# Autodesk Inventor assembly: Gripper
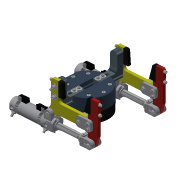
[picture p0: Inventor's stored thumbnail of the model, 180x180]
Saved by Autodesk Inventor 2020.1 (Build 241239000, 239)
## iProperties
Created: 2006-01-31
Part Number: Gripper
Document SubType Name: Assembly
Designer: Kevin
Manufacturer: Standard
Standards Organization: Custom
Weld Material: Default
Author: Kevin
Revision Number: -
## Documents named in this file (10)
- C:\Users\thomastremblay\Desktop\Inventor ACP Data\Gripper - References.iam
- C:\Users\thomastremblay\Desktop\Inventor ACP Data\Parts\210-100b.ipt
- C:\Users\thomastremblay\Desktop\Inventor ACP Data\Parts\210-101b.ipt
- C:\Users\thomastremblay\Desktop\Inventor ACP Data\Content Center\en-US\ISO 4762\M8-65.ipt
- C:\Users\thomastremblay\Desktop\Inventor ACP Data\Content Center\en-US\ISO 4762\M6-45.ipt
- C:\Users\thomastremblay\Desktop\Inventor ACP Data\Content Center\en-US\ISO 7089\10.ipt
- C:\Users\thomastremblay\Desktop\Inventor ACP Data\Content Center\en-US\ISO 4762\M8-30.ipt
- C:\Users\thomastremblay\Desktop\Inventor ACP Data\Parts\210-102 fb.ipt
- C:\Users\thomastremblay\Desktop\Inventor ACP Data\Assemblies\Clamp Assembly.iam
- C:\Users\thomastremblay\Desktop\Inventor ACP Data\Libraries\Simulation\Gripper_res_{3E676F27-C720-4572-8F7D-DA90B4A1A400}.fres
## Components (28 placed, 8 different names)
1. 210-100b:1 — Mate:1, Insert:1
2. 210-101b:1 — Mate:1, Insert:1, Mate:2, Mate:6, Mate:25, Mate:26, Mate:27, Mate:28, Mate:29, Insert:21, Mate:36, Mate:37, Mate:38, Mate:3
3. 210-102 fb:1 — Mate:2, Mate:3, Mate:42
4. 210-102 fb:2 — Mate:25, Mate:26, Mate:29, Mate:41, Rigid:1
5. Clamp Assembly:1 [sub-assembly]
6. Clamp Assembly:2 [sub-assembly] — Rigid:1
7. ISO 4762 M8 x 45:1 — Mate:6, Insert:22, Mate:42
8. ISO 7089 10 - 140 HV:1 — Insert:22
9. ISO 7089 10 - 140 HV:2 — Insert:23
10. ISO 4762 M8 x 45:2 — Insert:23, Mate:36
11. ISO 7089 10 - 140 HV:3 — Mate:28, Insert:25
12. ISO 4762 M8 x 45:3 — Insert:25, Mate:38
13. ISO 7089 10 - 140 HV:4 — Mate:27, Insert:24
14. ISO 4762 M8 x 45:4 — Mate:37, Insert:24
15. ISO 7089 10 - 140 HV:5 — Insert:33
16. ISO 7089 10 - 140 HV:6 — Insert:32
17. ISO 7089 10 - 140 HV:7 — Insert:28
18. ISO 7089 10 - 140 HV:8 — Insert:29
19. ISO 4762 M8 x 30:1 — Insert:29
20. ISO 4762 M8 x 30:2 — Insert:28, Mate:41
21. ISO 4762 M8 x 30:3 — Insert:32
22. ISO 4762 M8 x 30:4 — Insert:33
23. "ISO 4762 " M8 x 65:1 — Insert:21
24. "ISO 4762 " M8 x 65:2
25. "ISO 4762 " M8 x 65:3
26. "ISO 4762 " M8 x 65:4
27. "ISO 4762 " M8 x 65:5
28. "ISO 4762 " M8 x 65:6
## Component patterns: (8 elements, first: "ISO 4762 " M8 x 65:1)
## Relationships (33: Mate 17, Insert 14, Angle 1, WeldJoint 1)
- Mate:1: 210-100b:1 ↔ 210-101b:1
- Insert:1: 210-100b:1 ↔ 210-101b:1
- Mate:2: 210-101b:1 ↔ 210-102 fb:1
- [Mate]: 210-101b:1 ↔ 210-102 fb:1
- Mate:6: 210-101b:1 ↔ ISO 4762 M8 x 45:1
- [Mate]: 210-102 fb:2 ↔ ISO 7089 10 - 140 HV:1
- [Mate]: 210-101b:1 ↔ ISO 7089 10 - 140 HV:2
- Mate:25: 210-101b:1 ↔ 210-102 fb:2
- Mate:26: 210-101b:1 ↔ 210-102 fb:2
- Mate:27: 210-101b:1 ↔ ISO 7089 10 - 140 HV:4
- Mate:28: 210-101b:1 ↔ ISO 7089 10 - 140 HV:3
- Mate:29 (30 mm): 210-101b:1 ↔ 210-102 fb:2
- Insert:21: 210-101b:1 ↔ "ISO 4762 " M8 x 65:1
- Insert:22: ISO 4762 M8 x 45:1 ↔ ISO 7089 10 - 140 HV:1
- Insert:23: ISO 7089 10 - 140 HV:2 ↔ ISO 4762 M8 x 45:2
- Mate:36: 210-101b:1 ↔ ISO 4762 M8 x 45:2
- Mate:37: 210-101b:1 ↔ ISO 4762 M8 x 45:4
- Insert:24: ISO 7089 10 - 140 HV:4 ↔ ISO 4762 M8 x 45:4
- Insert:25: ISO 7089 10 - 140 HV:3 ↔ ISO 4762 M8 x 45:3
- Mate:38: 210-101b:1 ↔ ISO 4762 M8 x 45:3
- Insert:28: ISO 7089 10 - 140 HV:7 ↔ ISO 4762 M8 x 30:2
- Insert:29: ISO 7089 10 - 140 HV:8 ↔ ISO 4762 M8 x 30:1
- [Insert]: Clamp Assembly:1 ↔ ISO 7089 10 - 140 HV:6
- Insert:32: ISO 7089 10 - 140 HV:6 ↔ ISO 4762 M8 x 30:3
- Insert:33: ISO 7089 10 - 140 HV:5 ↔ ISO 4762 M8 x 30:4
- [Insert]: Clamp Assembly:1 ↔ ISO 7089 10 - 140 HV:5
- Mate:3: 210-101b:1 ↔ 210-102 fb:1
- [Insert]: 210-102 fb:1 ↔ Clamp Assembly:1
- [Angle] (0 deg): 210-102 fb:1 ↔ Clamp Assembly:1
- Mate:41: 210-102 fb:2 ↔ ISO 4762 M8 x 30:2
- Mate:42: 210-102 fb:1 ↔ ISO 4762 M8 x 45:1
- [Insert]: 210-102 fb:1 ↔ Clamp Assembly:1
- Rigid:1 [WeldJoint]: 210-102 fb:2 ↔ Clamp Assembly:2
## Named parameters: sa_0 = -1.46e-11, sa_1 = 14942.9, sa_2 = -1307.34, sa_3 = -1.68e-11, sa_4 = 14942.9, sa_5 = -1307.34, sa_6 = 427.41, sa_7 = -14502, sa_8 = -3809.04, sa_9 = 427.41, sa_10 = -14502, sa_11 = -3809.04, sa_12 = 712.349, sa_13 = -24170, sa_14 = -6348.39, sa_15 = -0, sa_16 = 24904.9, sa_17 = -2178.89
note: some values were not read from the file. Shown as the stored number, unit unknown: "sa_0", "sa_1", "sa_2", "sa_3", "sa_4", "sa_5", "sa_6", "sa_7", "sa_8", "sa_9", "sa_10", "sa_11", "sa_12", "sa_13", "sa_14", "sa_15", "sa_16", "sa_17".
